# Autodesk Inventor assembly: Suction stage with Module PCB
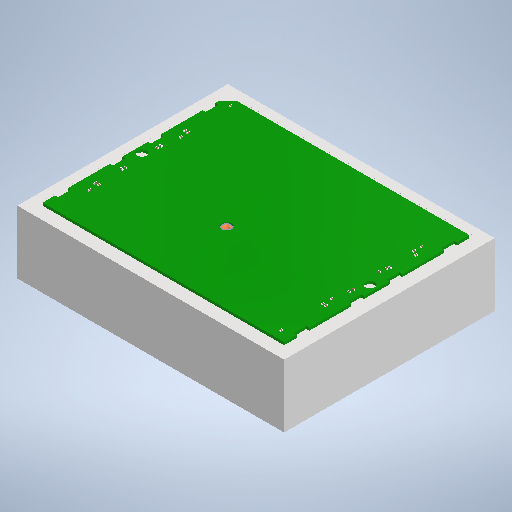
[picture p0: Inventor's stored thumbnail of the model, 512x512]
Saved by Autodesk Inventor 2025 (Build 290162000, 162)
## iProperties
Created: 2024-01-02
Part Number: Suction stage with Module PCB
Document SubType Name: Assembly
Designer: cfang
Author: cfang
## Documents named in this file (3)
- C:\Users\cfang\Desktop\nebraska-silicon-lab\Hardware\ETL\Module Assembly\Suction Stage V1\Suction stage with Module PCB.iam
- C:\Users\cfang\Desktop\nebraska-silicon-lab\Hardware\ETL\Module Assembly\Suction Stage V1\Suction Stage V1.ipt
- C:\Users\cfang\Desktop\nebraska-silicon-lab\Hardware\ETL\modules\tamale v1.5\Module PCB V1b\Module PCB V1b.ipt
## Components (2 placed, 2 different names)
1. Suction Stage V1:1 — Mate:1, Mate:2, Mate:3
2. Module PCB V1b:1 — Mate:1, Mate:2, Mate:3
## Relationships (3: Mate 3)
- Mate:1: Suction Stage V1:1 ↔ Module PCB V1b:1
- Mate:2 (1 mm): Suction Stage V1:1 ↔ Module PCB V1b:1
- Mate:3 (1 mm): Suction Stage V1:1 ↔ Module PCB V1b:1
